# Autodesk Inventor assembly: SISTEMA MOTRIZ
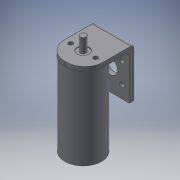
[picture p0: Inventor's stored thumbnail of the model, 180x180]
Saved by Autodesk Inventor 2019 (Build 230136000, 136)
## iProperties
Created: 2020-03-13
Part Number: SISTEMA MOTRIZ
Document SubType Name: Assembly
Designer: Hugo Albarracin
Author: Hugo Albarracin
## Documents named in this file (3)
- C:\Users\Hugo Albarracin\OneDrive - Escuela Superior Politécnica del Litoral\MECATRONICA UPM HUGO\14. TFM\iris_mecanico\sistema_motriz\SISTEMA MOTRIZ 3.iam
- C:\Users\Hugo Albarracin\OneDrive - Escuela Superior Politécnica del Litoral\MECATRONICA UPM HUGO\14. TFM\iris_mecanico\sistema_motriz\motor.ipt
- C:\Users\Hugo Albarracin\OneDrive - Escuela Superior Politécnica del Litoral\MECATRONICA UPM HUGO\14. TFM\iris_mecanico\sistema_motriz\soporte motor.ipt
## Components (2 placed, 2 different names)
1. motor:1 — Flush:1, Flush:2, Flush:3, Mate:1, Angle:1, Mate:2
2. soporte motor:1 — Mate:1, Angle:1, Mate:2
## Relationships (6: Flush 3, Mate 2, Angle 1)
- Flush:1: motor:1
- Flush:2: motor:1
- Flush:3: motor:1
- Mate:1: motor:1 ↔ soporte motor:1
- Angle:1 (0 deg): motor:1 ↔ soporte motor:1
- Mate:2: motor:1 ↔ soporte motor:1
